# Autodesk Inventor assembly: Serwo_z_widelcem
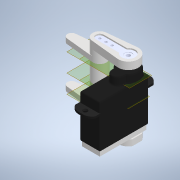
[picture p0: Inventor's stored thumbnail of the model, 180x180]
Saved by Autodesk Inventor 2022 (Build 260153000, 153)
## iProperties
Created: 2023-01-03
Part Number: Serwo_z_widelcem
Document SubType Name: Assembly
Designer: Kamil
Author: Kamil
## Documents named in this file (5)
- C:\MiniSumo koks\Serwo_z_widelcem.iam
- C:\MiniSumo koks\servo_mini_1370hd_cos.ipt
- C:\Users\Kamil\Downloads\servo horn.ipt
- C:\MiniSumo koks\Part6.ipt
- C:\MiniSumo koks\widelec.ipt
## Components (4 placed, 4 different names)
1. servo_mini_1370hd_cos:1 — Mate:1, Mate:2, Flush:1
2. servo horn:1 — Mate:1, Mate:2, Flush:2
3. Part6:1 — Flush:1
4. widelec:1 — Flush:2, Flush:3, Flush:6
## Relationships (8: Flush 6, Mate 2)
- Mate:1: servo_mini_1370hd_cos:1 ↔ servo horn:1
- Mate:2 (0.1 mm): servo_mini_1370hd_cos:1 ↔ servo horn:1
- Flush:1: servo_mini_1370hd_cos:1 ↔ Part6:1
- Flush:2: servo horn:1 ↔ widelec:1
- Flush:3 (-15 mm): widelec:1
- Flush:4 (7.5 mm)
- Flush:5 (-7.5 mm)
- Flush:6: widelec:1
